# Autodesk Inventor assembly: ReleaseAssembly
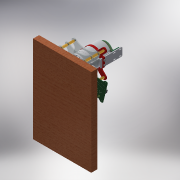
[picture p0: Inventor's stored thumbnail of the model, 180x180]
Saved by Autodesk Inventor 2018.2 (Build 222227000, 227)
## iProperties
Created: 2018-03-27
Part Number: ReleaseAssembly
Document SubType Name: Assembly
Designer: mansu
Author: mansu
## Documents named in this file (5)
- C:\Users\Moochster\OneDrive\Documents\2018 UBC\ELEC 391\Controller\cad\release\ReleaseAssembly.iam
- C:\Users\Moochster\OneDrive\Documents\2018 UBC\ELEC 391\Controller\cad\release\PitchAssembly.iam
- C:\Users\Moochster\OneDrive\Documents\2018 UBC\ELEC 391\Controller\cad\release\YawAssembly.iam
- C:\Users\Moochster\OneDrive\Documents\2018 UBC\ELEC 391\Controller\cad\release\WoodBase.ipt
- C:\Users\Moochster\OneDrive\Documents\2018 UBC\ELEC 391\Controller\cad\release\pcb.iam
## Components (4 placed, 4 different names)
1. PitchAssembly:1 [sub-assembly] — Flush:1, Mate:2
2. YawAssembly:1 [sub-assembly] — Mate:1, Flush:1
3. WoodBase:1 — Mate:2
4. pcb:1 [sub-assembly]
## Relationships (3: Mate 2, Flush 1)
- Mate:1: YawAssembly:1
- Flush:1: PitchAssembly:1 ↔ YawAssembly:1
- Mate:2: PitchAssembly:1 ↔ WoodBase:1
